# Autodesk Inventor assembly: 30-00 Injectomat suplimentar
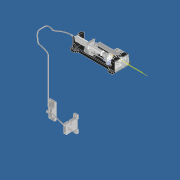
[picture p0: Inventor's stored thumbnail of the model, 180x180]
Saved by Autodesk Inventor 2020 (Build 240168000, 168)
## iProperties
Created: 2021-05-20
Part Number: 30-00 Injectomat suplimentar
Document SubType Name: Assembly
Designer: Iulian Bors
Author: Iulian Bors
## Documents named in this file (45)
- Z:\I.A.B\Proiecte\0008 I.A.B 3D 2.1 Imprimanta aracet Metal\30 Injectomat\30-00 Injectomat suplimentar.iam
- Z:\I.A.B\Proiecte\0008 I.A.B 3D 2.1 Imprimanta aracet Metal\30 Injectomat\syringe-100ml-1.snapshot.1\Corp.ipt
- Z:\I.A.B\Proiecte\0008 I.A.B 3D 2.1 Imprimanta aracet Metal\30 Injectomat\syringe-100ml-1.snapshot.1\Cauciuc.ipt
- Z:\I.A.B\Proiecte\0008 I.A.B 3D 2.1 Imprimanta aracet Metal\30 Injectomat\syringe-100ml-1.snapshot.1\Syringe_100ml.ipt
- Z:\I.A.B\Proiecte\0008 I.A.B 3D 2.1 Imprimanta aracet Metal\30 Injectomat\0008-30-002 Corp_Injectomat1.ipt
- Z:\I.A.B\Proiecte\0008 I.A.B 3D 2.1 Imprimanta aracet Metal\30 Injectomat\0008-30-001.ipt
- Z:\I.A.B\Proiecte\0008 I.A.B 3D 2.1 Imprimanta aracet Metal\30 Injectomat\0008-30-004.ipt
- Z:\I.A.B\Proiecte\0008 I.A.B 3D 2.1 Imprimanta aracet Metal\30 Injectomat\0008-30-1000 LMK8LUU.ipt
- Z:\I.A.B\Proiecte\0008 I.A.B 3D 2.1 Imprimanta aracet Metal\30 Injectomat\0008-30-1007 Bara 8.ipt
- Z:\I.A.B\Proiecte\0008 I.A.B 3D 2.1 Imprimanta aracet Metal\30 Injectomat\0008-30-1006 SHF8.ipt
- Z:\I.A.B\Proiecte\0008 I.A.B 3D 2.1 Imprimanta aracet Metal\30 Injectomat\0008-30-005.ipt
- Z:\I.A.B\Proiecte\0008 I.A.B 3D 2.1 Imprimanta aracet Metal\30 Injectomat\0008-30-1001 NEMA17 - Motor de passo.ipt
- Z:\I.A.B\Proiecte\0008 I.A.B 3D 2.1 Imprimanta aracet Metal\30 Injectomat\0008-30-1004 Piulita.ipt
- Z:\I.A.B\Proiecte\0008 I.A.B 3D 2.1 Imprimanta aracet Metal\30 Injectomat\0008-30-1003 T8 screw.ipt
- Z:\I.A.B\Proiecte\0008 I.A.B 3D 2.1 Imprimanta aracet Metal\30 Injectomat\0008-30-015 roata condusa GT2.ipt
- Z:\I.A.B\Proiecte\0008 I.A.B 3D 2.1 Imprimanta aracet Metal\30 Injectomat\0008-30-1011 GT2 Timing Pulley 20 Tooth.ipt
- Z:\I.A.B\Proiecte\0008 I.A.B 3D 2.1 Imprimanta aracet Metal\30 Injectomat\0008-30-1012 16T W6 B3 Without T_Shrinkwrap_1.ipt
- Z:\I.A.B\Proiecte\0008 I.A.B 3D 2.1 Imprimanta aracet Metal\30 Injectomat\0008-30-006.ipt
- Z:\I.A.B\Proiecte\0008 I.A.B 3D 2.1 Imprimanta aracet Metal\30 Injectomat\0008-30-1005 ISO 1224-1 - 10 - 8 x 22 x 7.ipt
- Z:\I.A.B\Proiecte\0008 I.A.B 3D 2.1 Imprimanta aracet Metal\30 Injectomat\I.A.B 2.1 Aracet_Subansamble_Shrinkwrap_2.ipt
- Z:\I.A.B\Proiecte\0008 I.A.B 3D 2.1 Imprimanta aracet Metal\30 Injectomat\0008-30-007.ipt
- Z:\I.A.B\Proiecte\0008 I.A.B 3D 2.1 Imprimanta aracet Metal\30 Injectomat\0008-30-008.ipt
- Z:\I.A.B\Proiecte\0008 I.A.B 3D 2.1 Imprimanta aracet Metal\30 Injectomat\0008-30-2002 DIN 125 - A 4.3.ipt
- Z:\I.A.B\Proiecte\0008 I.A.B 3D 2.1 Imprimanta aracet Metal\30 Injectomat\0008-30-2019 DIN 6912 - M4 x 50.ipt
- Z:\I.A.B\Proiecte\0008 I.A.B 3D 2.1 Imprimanta aracet Metal\30 Injectomat\0008-30-009.ipt
- Z:\I.A.B\Proiecte\0008 I.A.B 3D 2.1 Imprimanta aracet Metal\30 Injectomat\0008-30-2016 DIN 315 - M4.ipt
- Z:\I.A.B\Proiecte\0008 I.A.B 3D 2.1 Imprimanta aracet Metal\30 Injectomat\0008-30-010.ipt
- Z:\I.A.B\Proiecte\0008 I.A.B 3D 2.1 Imprimanta aracet Metal\30 Injectomat\0008-30-011.ipt
- Z:\I.A.B\Proiecte\0008 I.A.B 3D 2.1 Imprimanta aracet Metal\30 Injectomat\0008-30-1008 Adaptor furtun.ipt
- Z:\I.A.B\Proiecte\0008 I.A.B 3D 2.1 Imprimanta aracet Metal\30 Injectomat\0008-30-012.ipt
- Z:\I.A.B\Proiecte\0008 I.A.B 3D 2.1 Imprimanta aracet Metal\30 Injectomat\0008-30-1009 Adaptor Ac.ipt
- Z:\I.A.B\Proiecte\0008 I.A.B 3D 2.1 Imprimanta aracet Metal\30 Injectomat\0008-30-013.ipt
- Z:\I.A.B\Proiecte\0008 I.A.B 3D 2.1 Imprimanta aracet Metal\30 Injectomat\0008-30-014.ipt
- Z:\I.A.B\Proiecte\0008 I.A.B 3D 2.1 Imprimanta aracet Metal\10 Mecanic\Seringa\syringe-57.snapshot.2\SYRINGE (INVENTOR)\Needle.ipt
- Z:\I.A.B\Proiecte\0008 I.A.B 3D 2.1 Imprimanta aracet Metal\30 Injectomat\0008-30-2001 DIN 934 - M4 x 0.7.ipt
- Z:\I.A.B\Proiecte\0008 I.A.B 3D 2.1 Imprimanta aracet Metal\30 Injectomat\0008-30-203 DIN 7991 - M4x20.ipt
- Z:\I.A.B\Proiecte\0008 I.A.B 3D 2.1 Imprimanta aracet Metal\10 Mecanic\m3X16.iam
- Z:\I.A.B\Proiecte\0008 I.A.B 3D 2.1 Imprimanta aracet Metal\10 Mecanic\0008-10-2008 DIN 912 - M3 x 0.5 x 25 x 18.ipt
- Z:\I.A.B\Proiecte\0008 I.A.B 3D 2.1 Imprimanta aracet Metal\10 Mecanic\0008-10-2005 DIN 125 - A 3.2.ipt
- Z:\I.A.B\Proiecte\0008 I.A.B 3D 2.1 Imprimanta aracet Metal\10 Mecanic\0008-10-2009 DIN 555-5 - M3.ipt
- Z:\I.A.B\Proiecte\0008 I.A.B 3D 2.1 Imprimanta aracet Metal\10 Mecanic\0008-10-2004 DIN 7984 - M3 x 20.ipt
- Z:\I.A.B\Proiecte\0008 I.A.B 3D 2.1 Imprimanta aracet Metal\10 Mecanic\0008-10-2006 DIN 7984 - M3 x 16.ipt
- Z:\I.A.B\Proiecte\0008 I.A.B 3D 2.1 Imprimanta aracet Metal\30 Injectomat\30-00 Injectomat suplimentar\Design Accelerator\Synchronous Belts Transmission2.iam
- Z:\I.A.B\Proiecte\0008 I.A.B 3D 2.1 Imprimanta aracet Metal\10 Mecanic\SurubM4x25.iam
- Z:\I.A.B\Proiecte\0008 I.A.B 3D 2.1 Imprimanta aracet Metal\30 Injectomat\0008-30-2030 DIN EN ISO 4029 - M4  x  5.ipt
## Components (148 placed, 44 different names)
1. Corp.ipt:1 — Mate:1, Flush:3, Mate:18, Tangent:1, Insert:15
2. Cauciuc.ipt:2 — Insert:1, Mate:1, Mate:17
3. Syringe_100ml.ipt:3 — Insert:1, Angle:1, Mate:4, Mate:5
4. 0008-30-002 Corp_Injectomat1.ipt:4 — Angle:2, Angle:3, Angle:4, Angle:6, Mate:10, Mate:12, Mate:18, Mate:27, Tangent:1, Mate:34, Flush:8, Mate:38, Insert:6, Mate:44, Mate:45, Mate:46, Mate:47, Mate:48, Flush:10, Flush:18, Insert:27, Insert:38, Insert:39, Insert:40, Insert:41, Insert:42, Tangent:2, Insert:99, Insert:100, Insert:103, Insert:104
5. 0008-30-001.ipt:5 — Angle:3, Angle:4, Insert:3, Mate:20, Flush:6, Flush:7, Mate:21, Mate:23, Mate:24, Mate:25, Insert:64, Insert:74, Insert:75, Insert:76
6. 0008-30-004.ipt:6 — Insert:3, Mate:4, Mate:5
7. 0008-30-1000 LMK8LUU.ipt:7 — Mate:8, Mate:19, Flush:5, Flush:6, Flush:7, Mate:25, Insert:116, Insert:117, Insert:118, Insert:119
8. 0008-30-1000 LMK8LUU.ipt:8 — Mate:9, Mate:19, Mate:20, Flush:5, Insert:120, Insert:121, Insert:122, Insert:124
9. 0008-30-1007 Bara 8.ipt:9 — Mate:8, Flush:2, Mate:39, Mate:41
10. 0008-30-1007 Bara 8.ipt:10 — Mate:9, Flush:1, Mate:33, Mate:42
11. 0008-30-1006 SHF8.ipt:11 — Angle:6, Flush:2, Mate:38, Mate:39, Insert:60, Insert:93, Insert:94
12. 0008-30-1006 SHF8.ipt:12 — Flush:1, Mate:33, Mate:34, Insert:56, Insert:95, Insert:96
13. 0008-30-005.ipt:13 — Mate:10, Flush:3, Mate:17, Mate:43, Insert:10, Insert:13
14. I.A.B 2.1 Aracet_Subansamble_Shrinkwrap_2.ipt:14 — Mate:49, Flush:11, Mate:50, Flush:16, Flush:17, Flush:18, Mate:52
15. 0008-30-1001 NEMA17 - Motor de passo.ipt:15 — Mate:12, Insert:4, Flush:8, Tangent:2, Insert:86, Insert:90, Insert:91, Insert:92
16. 0008-30-1004 Piulita.ipt:16 — Mate:21, Mate:22, Mate:23, Mate:24, Insert:78, Insert:82, Insert:83, Insert:84
17. 0008-30-1003 T8 screw.ipt:17 — Mate:22, Mate:26, Flush:9, Insert:5, Mate:59
18. 0008-30-015 roata condusa GT2.ipt:18 — Mate:26, Mate:27, Flush:9, Mate:56
19. 0008-30-1011 GT2 Timing Pulley 20 Tooth.ipt:19 — Insert:4, Mate:55, Mate:57
20. 0008-30-1012 16T W6 B3 Without T_Shrinkwrap_1.ipt:20 — Mate:53, Mate:54
21. 0008-30-006.ipt:21 — Mate:41, Mate:42, Mate:43, Insert:49, Insert:50, Insert:51, Insert:52
22. 0008-30-1005 ISO 1224-1 - 10 - 8 x 22 x 7.ipt:22 — Insert:5, Insert:14
23. 0008-30-1005 ISO 1224-1 - 10 - 8 x 22 x 7.ipt:23 — Insert:6, Insert:8
24. 0008-30-007.ipt:24 — Mate:53, Mate:54
25. 0008-30-008.ipt:25 — Insert:8, Mate:58
26. 0008-30-2002 DIN 125 - A 4.3.ipt:26 — Insert:9, Insert:10
27. 0008-30-2019 DIN 6912 - M4 x 50.ipt:27 — Insert:9, Insert:12
28. 0008-30-009.ipt:28 — Insert:13
29. 0008-30-2016 DIN 315 - M4.ipt:29 — Insert:12
30. 0008-30-008.ipt:30 — Insert:14
31. 0008-30-010.ipt:31 — Mate:44, Mate:45, Mate:46
32. 0008-30-011.ipt:32 — Mate:47, Mate:48, Flush:10
33. 0008-30-2002 DIN 125 - A 4.3.ipt:33 — Insert:17, Insert:20
34. 0008-30-1008 Adaptor furtun.ipt:34 — Insert:15
35. 0008-30-012.ipt:35 — Mate:49, Flush:11, Flush:12, Flush:13, Mate:51, Flush:14, Flush:15
36. 0008-30-1009 Adaptor Ac.ipt:36 — Flush:12, Mate:50, Flush:13, Insert:16
37. 0008-30-013.ipt:37 — Mate:51, Flush:14, Flush:15, Insert:20, Insert:24
38. 0008-30-014.ipt:38 — Flush:16, Flush:17, Mate:52
39. Needle.ipt:39 — Insert:16
40. 0008-30-2001 DIN 934 - M4 x 0.7.ipt:40 — Insert:18, Insert:19
41. 0008-30-2019 DIN 6912 - M4 x 50.ipt:41 — Insert:17, Insert:19
42. 0008-30-2002 DIN 125 - A 4.3.ipt:42 — Insert:18
43. 0008-30-2001 DIN 934 - M4 x 0.7.ipt:43
44. 0008-30-2002 DIN 125 - A 4.3.ipt:44 — Insert:24
45. 0008-30-2019 DIN 6912 - M4 x 50.ipt:45
46. 0008-30-2002 DIN 125 - A 4.3.ipt:46
47. 0008-30-203 DIN 7991 - M4x20.ipt:47 — Insert:26, Insert:27
48. 0008-30-2001 DIN 934 - M4 x 0.7.ipt:48 — Insert:26
49. 0008-30-2002 DIN 125 - A 4.3.ipt:49
50. 0008-30-203 DIN 7991 - M4x20.ipt:50 — Insert:42
51. 0008-30-2001 DIN 934 - M4 x 0.7.ipt:51
52. 0008-30-2002 DIN 125 - A 4.3.ipt:52
53. 0008-30-203 DIN 7991 - M4x20.ipt:53 — Insert:41
54. 0008-30-2001 DIN 934 - M4 x 0.7.ipt:54
55. 0008-30-2002 DIN 125 - A 4.3.ipt:55
56. 0008-30-203 DIN 7991 - M4x20.ipt:56 — Insert:40
57. 0008-30-2001 DIN 934 - M4 x 0.7.ipt:57
58. 0008-30-2002 DIN 125 - A 4.3.ipt:58
59. 0008-30-203 DIN 7991 - M4x20.ipt:59 — Insert:38
60. 0008-30-2001 DIN 934 - M4 x 0.7.ipt:60
61. 0008-30-2002 DIN 125 - A 4.3.ipt:61
62. 0008-30-203 DIN 7991 - M4x20.ipt:62 — Insert:39
63. 0008-30-2001 DIN 934 - M4 x 0.7.ipt:63
64. 0008-30-2002 DIN 125 - A 4.3.ipt:64
65. 0008-30-2001 DIN 934 - M4 x 0.7.ipt:65
66. 0008-30-2002 DIN 125 - A 4.3.ipt:66 — Insert:50
67. 0008-30-2019 DIN 6912 - M4 x 50.ipt:67
68. 0008-30-2002 DIN 125 - A 4.3.ipt:68
69. 0008-30-2001 DIN 934 - M4 x 0.7.ipt:69
70. 0008-30-2002 DIN 125 - A 4.3.ipt:70 — Insert:49
71. 0008-30-2019 DIN 6912 - M4 x 50.ipt:71
72. 0008-30-2002 DIN 125 - A 4.3.ipt:72
73. m3X16.iam:73 [sub-assembly] — Insert:51
74. m3X16.iam:74 [sub-assembly] — Insert:52
75. 0008-10-2008 DIN 912 - M3 x 0.5 x 25 x 18.ipt:75 — Insert:53, Insert:55
76. 0008-10-2005 DIN 125 - A 3.2.ipt:76 — Insert:54
77. 0008-10-2009 DIN 555-5 - M3.ipt:77 — Insert:54, Insert:55
78. 0008-10-2005 DIN 125 - A 3.2.ipt:78 — Insert:53, Insert:56
79. 0008-10-2008 DIN 912 - M3 x 0.5 x 25 x 18.ipt:79
80. 0008-10-2005 DIN 125 - A 3.2.ipt:80
81. 0008-10-2009 DIN 555-5 - M3.ipt:81
82. 0008-10-2005 DIN 125 - A 3.2.ipt:82 — Insert:60
83. 0008-10-2009 DIN 555-5 - M3.ipt:83 — Insert:63
84. 0008-10-2005 DIN 125 - A 3.2.ipt:84
85. 0008-10-2005 DIN 125 - A 3.2.ipt:85 — Insert:62, Insert:64
86. 0008-10-2004 DIN 7984 - M3 x 20.ipt:86 — Insert:62, Insert:63
87. 0008-10-2009 DIN 555-5 - M3.ipt:87
88. 0008-10-2005 DIN 125 - A 3.2.ipt:88
89. 0008-10-2005 DIN 125 - A 3.2.ipt:89 — Insert:76
90. 0008-10-2004 DIN 7984 - M3 x 20.ipt:90
91. 0008-10-2009 DIN 555-5 - M3.ipt:91
92. 0008-10-2005 DIN 125 - A 3.2.ipt:92
93. 0008-10-2005 DIN 125 - A 3.2.ipt:93 — Insert:75
94. 0008-10-2004 DIN 7984 - M3 x 20.ipt:94
95. 0008-10-2009 DIN 555-5 - M3.ipt:95
96. 0008-10-2005 DIN 125 - A 3.2.ipt:96
97. 0008-10-2005 DIN 125 - A 3.2.ipt:97 — Insert:74
98. 0008-10-2004 DIN 7984 - M3 x 20.ipt:98
99. 0008-10-2006 DIN 7984 - M3 x 16.ipt:99 — Insert:78
100. 0008-10-2009 DIN 555-5 - M3.ipt:100
101. 0008-10-2006 DIN 7984 - M3 x 16.ipt:101 — Insert:82
102. 0008-10-2009 DIN 555-5 - M3.ipt:102
103. 0008-10-2006 DIN 7984 - M3 x 16.ipt:103 — Insert:83
104. 0008-10-2009 DIN 555-5 - M3.ipt:104
105. 0008-10-2006 DIN 7984 - M3 x 16.ipt:105 — Insert:84
106. 0008-10-2009 DIN 555-5 - M3.ipt:106
107. Synchronous Belts Transmission2.iam:107 [sub-assembly] — Mate:55, Mate:56, Mate:57
108. 0008-10-2006 DIN 7984 - M3 x 16.ipt:108
109. 0008-10-2005 DIN 125 - A 3.2.ipt:109 — Insert:86
110. 0008-10-2006 DIN 7984 - M3 x 16.ipt:110
111. 0008-10-2005 DIN 125 - A 3.2.ipt:111 — Insert:90
112. 0008-10-2006 DIN 7984 - M3 x 16.ipt:112
113. 0008-10-2005 DIN 125 - A 3.2.ipt:113 — Insert:92
114. 0008-10-2006 DIN 7984 - M3 x 16.ipt:114
115. 0008-10-2005 DIN 125 - A 3.2.ipt:115 — Insert:91
116. SurubM4x25.iam:116 [sub-assembly] — Insert:93
117. SurubM4x25.iam:117 [sub-assembly] — Insert:95
118. SurubM4x25.iam:118 [sub-assembly] — Insert:94
119. SurubM4x25.iam:119 [sub-assembly] — Insert:96
120. 0008-10-2005 DIN 125 - A 3.2.ipt:120 — Insert:99
121. 0008-10-2004 DIN 7984 - M3 x 20.ipt:121 — Insert:107
122. 0008-10-2005 DIN 125 - A 3.2.ipt:122 — Insert:100
123. 0008-10-2004 DIN 7984 - M3 x 20.ipt:123 — Insert:108
124. 0008-10-2009 DIN 555-5 - M3.ipt:124
125. 0008-10-2005 DIN 125 - A 3.2.ipt:125 — Insert:103
126. 0008-10-2009 DIN 555-5 - M3.ipt:126
127. 0008-10-2005 DIN 125 - A 3.2.ipt:127 — Insert:104
128. 0008-10-2009 DIN 555-5 - M3.ipt:128 — Insert:107
129. 0008-10-2005 DIN 125 - A 3.2.ipt:129
130. 0008-10-2009 DIN 555-5 - M3.ipt:130 — Insert:108
131. 0008-10-2005 DIN 125 - A 3.2.ipt:131
132. 0008-10-2006 DIN 7984 - M3 x 16.ipt:132 — Insert:117
133. 0008-10-2009 DIN 555-5 - M3.ipt:133
134. 0008-10-2006 DIN 7984 - M3 x 16.ipt:134 — Insert:118
135. 0008-10-2009 DIN 555-5 - M3.ipt:135
136. 0008-10-2006 DIN 7984 - M3 x 16.ipt:136 — Insert:119
137. 0008-10-2009 DIN 555-5 - M3.ipt:137
138. 0008-10-2006 DIN 7984 - M3 x 16.ipt:138 — Insert:121
139. 0008-10-2009 DIN 555-5 - M3.ipt:139
140. 0008-10-2006 DIN 7984 - M3 x 16.ipt:140 — Insert:122
141. 0008-10-2009 DIN 555-5 - M3.ipt:141
142. 0008-10-2006 DIN 7984 - M3 x 16.ipt:142 — Insert:120
143. 0008-10-2009 DIN 555-5 - M3.ipt:143
144. 0008-10-2006 DIN 7984 - M3 x 16.ipt:144 — Insert:116
145. 0008-10-2009 DIN 555-5 - M3.ipt:145
146. 0008-10-2006 DIN 7984 - M3 x 16.ipt:146 — Insert:124
147. 0008-10-2009 DIN 555-5 - M3.ipt:147
148. 0008-30-2030 DIN EN ISO 4029 - M4  x  5.ipt:148 — Mate:58, Mate:59
## Relationships (188: Insert 121, Mate 42, Flush 18, Angle 5, Tangent 2)
- Insert:1: Cauciuc.ipt:2 ↔ Syringe_100ml.ipt:3
- Mate:1: Corp.ipt:1 ↔ Cauciuc.ipt:2
- Angle:1 (0 deg): Syringe_100ml.ipt:3
- Angle:2 (180 deg): 0008-30-002 Corp_Injectomat1.ipt:4
- Angle:3 (180 deg): 0008-30-002 Corp_Injectomat1.ipt:4 ↔ 0008-30-001.ipt:5
- Angle:4 (180 deg): 0008-30-002 Corp_Injectomat1.ipt:4 ↔ 0008-30-001.ipt:5
- Insert:3: 0008-30-001.ipt:5 ↔ 0008-30-004.ipt:6
- Mate:4: Syringe_100ml.ipt:3 ↔ 0008-30-004.ipt:6
- Mate:5: Syringe_100ml.ipt:3 ↔ 0008-30-004.ipt:6
- Mate:8: 0008-30-1000 LMK8LUU.ipt:7 ↔ 0008-30-1007 Bara 8.ipt:9
- Mate:9: 0008-30-1000 LMK8LUU.ipt:8 ↔ 0008-30-1007 Bara 8.ipt:10
- Angle:6 (0 deg): 0008-30-002 Corp_Injectomat1.ipt:4 ↔ 0008-30-1006 SHF8.ipt:11
- Flush:1: 0008-30-1007 Bara 8.ipt:10 ↔ 0008-30-1006 SHF8.ipt:12
- Flush:2: 0008-30-1007 Bara 8.ipt:9 ↔ 0008-30-1006 SHF8.ipt:11
- [Flush] (30 mm): 0008-30-002 Corp_Injectomat1.ipt:4 ↔ I.A.B 2.1 Aracet_Subansamble_Shrinkwrap_2.ipt:14
- Mate:10: 0008-30-002 Corp_Injectomat1.ipt:4 ↔ 0008-30-005.ipt:13
- Flush:3 (-5 mm): Corp.ipt:1 ↔ 0008-30-005.ipt:13
- [Mate]: 0008-30-002 Corp_Injectomat1.ipt:4 ↔ I.A.B 2.1 Aracet_Subansamble_Shrinkwrap_2.ipt:14
- Mate:12: 0008-30-002 Corp_Injectomat1.ipt:4 ↔ 0008-30-1001 NEMA17 - Motor de passo.ipt:15
- Mate:17: Cauciuc.ipt:2 ↔ 0008-30-005.ipt:13
- Mate:18: Corp.ipt:1 ↔ 0008-30-002 Corp_Injectomat1.ipt:4
- Mate:19 (3 mm): 0008-30-1000 LMK8LUU.ipt:7 ↔ 0008-30-1000 LMK8LUU.ipt:8
- Mate:20: 0008-30-001.ipt:5 ↔ 0008-30-1000 LMK8LUU.ipt:8
- Flush:5: 0008-30-1000 LMK8LUU.ipt:7 ↔ 0008-30-1000 LMK8LUU.ipt:8
- Flush:6 (5 mm): 0008-30-001.ipt:5 ↔ 0008-30-1000 LMK8LUU.ipt:7
- Flush:7 (40 mm): 0008-30-001.ipt:5 ↔ 0008-30-1000 LMK8LUU.ipt:7
- Mate:21: 0008-30-001.ipt:5 ↔ 0008-30-1004 Piulita.ipt:16
- Mate:22: 0008-30-1004 Piulita.ipt:16 ↔ 0008-30-1003 T8 screw.ipt:17
- Mate:23: 0008-30-001.ipt:5 ↔ 0008-30-1004 Piulita.ipt:16
- Mate:24: 0008-30-001.ipt:5 ↔ 0008-30-1004 Piulita.ipt:16
- Mate:25: 0008-30-001.ipt:5 ↔ 0008-30-1000 LMK8LUU.ipt:7
- Mate:26: 0008-30-1003 T8 screw.ipt:17 ↔ 0008-30-015 roata condusa GT2.ipt:18
- Mate:27 (1 mm): 0008-30-002 Corp_Injectomat1.ipt:4 ↔ 0008-30-015 roata condusa GT2.ipt:18
- Tangent:1 (-0.5 mm): Corp.ipt:1 ↔ 0008-30-002 Corp_Injectomat1.ipt:4
- Insert:4 (2 mm): 0008-30-1001 NEMA17 - Motor de passo.ipt:15 ↔ 0008-30-1011 GT2 Timing Pulley 20 Tooth.ipt:19
- Mate:33: 0008-30-1007 Bara 8.ipt:10 ↔ 0008-30-1006 SHF8.ipt:12
- Mate:34: 0008-30-002 Corp_Injectomat1.ipt:4 ↔ 0008-30-1006 SHF8.ipt:12
- Flush:8 (1 mm): 0008-30-002 Corp_Injectomat1.ipt:4 ↔ 0008-30-1001 NEMA17 - Motor de passo.ipt:15
- Mate:38: 0008-30-002 Corp_Injectomat1.ipt:4 ↔ 0008-30-1006 SHF8.ipt:11
- Mate:39: 0008-30-1007 Bara 8.ipt:9 ↔ 0008-30-1006 SHF8.ipt:11
- Flush:9: 0008-30-1003 T8 screw.ipt:17 ↔ 0008-30-015 roata condusa GT2.ipt:18
- Mate:41: 0008-30-1007 Bara 8.ipt:9 ↔ 0008-30-006.ipt:21
- Mate:42: 0008-30-1007 Bara 8.ipt:10 ↔ 0008-30-006.ipt:21
- Mate:43: 0008-30-005.ipt:13 ↔ 0008-30-006.ipt:21
- Insert:5: 0008-30-1003 T8 screw.ipt:17 ↔ 0008-30-1005 ISO 1224-1 - 10 - 8 x 22 x 7.ipt:22
- Insert:6: 0008-30-002 Corp_Injectomat1.ipt:4 ↔ 0008-30-1005 ISO 1224-1 - 10 - 8 x 22 x 7.ipt:23
- Insert:8: 0008-30-1005 ISO 1224-1 - 10 - 8 x 22 x 7.ipt:23 ↔ 0008-30-008.ipt:25
- Insert:9: 0008-30-2002 DIN 125 - A 4.3.ipt:26 ↔ 0008-30-2019 DIN 6912 - M4 x 50.ipt:27
- Insert:10: 0008-30-005.ipt:13 ↔ 0008-30-2002 DIN 125 - A 4.3.ipt:26
- Insert:12: 0008-30-2019 DIN 6912 - M4 x 50.ipt:27 ↔ 0008-30-2016 DIN 315 - M4.ipt:29
- Insert:13: 0008-30-005.ipt:13 ↔ 0008-30-009.ipt:28
- Insert:14: 0008-30-1005 ISO 1224-1 - 10 - 8 x 22 x 7.ipt:22 ↔ 0008-30-008.ipt:30
- Mate:44: 0008-30-002 Corp_Injectomat1.ipt:4 ↔ 0008-30-010.ipt:31
- Mate:45 (1 mm): 0008-30-002 Corp_Injectomat1.ipt:4 ↔ 0008-30-010.ipt:31
- Mate:46 (1 mm): 0008-30-002 Corp_Injectomat1.ipt:4 ↔ 0008-30-010.ipt:31
- Mate:47: 0008-30-002 Corp_Injectomat1.ipt:4 ↔ 0008-30-011.ipt:32
- Mate:48: 0008-30-002 Corp_Injectomat1.ipt:4 ↔ 0008-30-011.ipt:32
- Flush:10: 0008-30-002 Corp_Injectomat1.ipt:4 ↔ 0008-30-011.ipt:32
- Insert:15: Corp.ipt:1 ↔ 0008-30-1008 Adaptor furtun.ipt:34
- Mate:49: I.A.B 2.1 Aracet_Subansamble_Shrinkwrap_2.ipt:14 ↔ 0008-30-012.ipt:35
- Flush:11: I.A.B 2.1 Aracet_Subansamble_Shrinkwrap_2.ipt:14 ↔ 0008-30-012.ipt:35
- Flush:12 (-2 mm): 0008-30-012.ipt:35 ↔ 0008-30-1009 Adaptor Ac.ipt:36
- Mate:50 (77 mm): I.A.B 2.1 Aracet_Subansamble_Shrinkwrap_2.ipt:14 ↔ 0008-30-1009 Adaptor Ac.ipt:36
- Flush:13: 0008-30-012.ipt:35 ↔ 0008-30-1009 Adaptor Ac.ipt:36
- Mate:51 (2 mm): 0008-30-012.ipt:35 ↔ 0008-30-013.ipt:37
- Flush:14: 0008-30-012.ipt:35 ↔ 0008-30-013.ipt:37
- Flush:15: 0008-30-012.ipt:35 ↔ 0008-30-013.ipt:37
- Flush:16: I.A.B 2.1 Aracet_Subansamble_Shrinkwrap_2.ipt:14 ↔ 0008-30-014.ipt:38
- Flush:17: I.A.B 2.1 Aracet_Subansamble_Shrinkwrap_2.ipt:14 ↔ 0008-30-014.ipt:38
- Flush:18 (-2 mm): 0008-30-002 Corp_Injectomat1.ipt:4 ↔ I.A.B 2.1 Aracet_Subansamble_Shrinkwrap_2.ipt:14
- Mate:52: I.A.B 2.1 Aracet_Subansamble_Shrinkwrap_2.ipt:14 ↔ 0008-30-014.ipt:38
- Insert:16 (-5 mm): 0008-30-1009 Adaptor Ac.ipt:36 ↔ Needle.ipt:39
- Mate:53: 0008-30-1012 16T W6 B3 Without T_Shrinkwrap_1.ipt:20 ↔ 0008-30-007.ipt:24
- Mate:54: 0008-30-1012 16T W6 B3 Without T_Shrinkwrap_1.ipt:20 ↔ 0008-30-007.ipt:24
- Insert:17: 0008-30-2002 DIN 125 - A 4.3.ipt:33 ↔ 0008-30-2019 DIN 6912 - M4 x 50.ipt:41
- Insert:18: 0008-30-2001 DIN 934 - M4 x 0.7.ipt:40 ↔ 0008-30-2002 DIN 125 - A 4.3.ipt:42
- Insert:19: 0008-30-2001 DIN 934 - M4 x 0.7.ipt:40 ↔ 0008-30-2019 DIN 6912 - M4 x 50.ipt:41
- Insert:20: 0008-30-2002 DIN 125 - A 4.3.ipt:33 ↔ 0008-30-013.ipt:37
- [Insert]: 0008-30-2002 DIN 125 - A 4.3.ipt:44 ↔ 0008-30-2019 DIN 6912 - M4 x 50.ipt:45
- [Insert]: 0008-30-2001 DIN 934 - M4 x 0.7.ipt:43 ↔ 0008-30-2002 DIN 125 - A 4.3.ipt:46
- [Insert]: 0008-30-2001 DIN 934 - M4 x 0.7.ipt:43 ↔ 0008-30-2019 DIN 6912 - M4 x 50.ipt:45
- Insert:24: 0008-30-013.ipt:37 ↔ 0008-30-2002 DIN 125 - A 4.3.ipt:44
- [Insert]: 0008-30-2001 DIN 934 - M4 x 0.7.ipt:48 ↔ 0008-30-2002 DIN 125 - A 4.3.ipt:49
- Insert:26: 0008-30-203 DIN 7991 - M4x20.ipt:47 ↔ 0008-30-2001 DIN 934 - M4 x 0.7.ipt:48
- Insert:27: 0008-30-002 Corp_Injectomat1.ipt:4 ↔ 0008-30-203 DIN 7991 - M4x20.ipt:47
- [Insert]: 0008-30-2001 DIN 934 - M4 x 0.7.ipt:51 ↔ 0008-30-2002 DIN 125 - A 4.3.ipt:52
- [Insert]: 0008-30-203 DIN 7991 - M4x20.ipt:50 ↔ 0008-30-2001 DIN 934 - M4 x 0.7.ipt:51
- [Insert]: 0008-30-2001 DIN 934 - M4 x 0.7.ipt:54 ↔ 0008-30-2002 DIN 125 - A 4.3.ipt:55
- [Insert]: 0008-30-203 DIN 7991 - M4x20.ipt:53 ↔ 0008-30-2001 DIN 934 - M4 x 0.7.ipt:54
- [Insert]: 0008-30-2001 DIN 934 - M4 x 0.7.ipt:57 ↔ 0008-30-2002 DIN 125 - A 4.3.ipt:58
- [Insert]: 0008-30-203 DIN 7991 - M4x20.ipt:56 ↔ 0008-30-2001 DIN 934 - M4 x 0.7.ipt:57
- [Insert]: 0008-30-2001 DIN 934 - M4 x 0.7.ipt:60 ↔ 0008-30-2002 DIN 125 - A 4.3.ipt:61
- [Insert]: 0008-30-203 DIN 7991 - M4x20.ipt:59 ↔ 0008-30-2001 DIN 934 - M4 x 0.7.ipt:60
- [Insert]: 0008-30-2001 DIN 934 - M4 x 0.7.ipt:63 ↔ 0008-30-2002 DIN 125 - A 4.3.ipt:64
- [Insert]: 0008-30-203 DIN 7991 - M4x20.ipt:62 ↔ 0008-30-2001 DIN 934 - M4 x 0.7.ipt:63
- Insert:38: 0008-30-002 Corp_Injectomat1.ipt:4 ↔ 0008-30-203 DIN 7991 - M4x20.ipt:59
- Insert:39: 0008-30-002 Corp_Injectomat1.ipt:4 ↔ 0008-30-203 DIN 7991 - M4x20.ipt:62
- Insert:40: 0008-30-002 Corp_Injectomat1.ipt:4 ↔ 0008-30-203 DIN 7991 - M4x20.ipt:56
- Insert:41: 0008-30-002 Corp_Injectomat1.ipt:4 ↔ 0008-30-203 DIN 7991 - M4x20.ipt:53
- Insert:42: 0008-30-002 Corp_Injectomat1.ipt:4 ↔ 0008-30-203 DIN 7991 - M4x20.ipt:50
- [Insert]: 0008-30-2002 DIN 125 - A 4.3.ipt:66 ↔ 0008-30-2019 DIN 6912 - M4 x 50.ipt:67
- [Insert]: 0008-30-2001 DIN 934 - M4 x 0.7.ipt:65 ↔ 0008-30-2002 DIN 125 - A 4.3.ipt:68
- [Insert]: 0008-30-2001 DIN 934 - M4 x 0.7.ipt:65 ↔ 0008-30-2019 DIN 6912 - M4 x 50.ipt:67
- [Insert]: 0008-30-2002 DIN 125 - A 4.3.ipt:70 ↔ 0008-30-2019 DIN 6912 - M4 x 50.ipt:71
- [Insert]: 0008-30-2001 DIN 934 - M4 x 0.7.ipt:69 ↔ 0008-30-2002 DIN 125 - A 4.3.ipt:72
- [Insert]: 0008-30-2001 DIN 934 - M4 x 0.7.ipt:69 ↔ 0008-30-2019 DIN 6912 - M4 x 50.ipt:71
- Insert:49: 0008-30-006.ipt:21 ↔ 0008-30-2002 DIN 125 - A 4.3.ipt:70
- Insert:50: 0008-30-006.ipt:21 ↔ 0008-30-2002 DIN 125 - A 4.3.ipt:66
- Insert:51: 0008-30-006.ipt:21 ↔ m3X16.iam:73
- Insert:52: 0008-30-006.ipt:21 ↔ m3X16.iam:74
- Insert:53: 0008-10-2008 DIN 912 - M3 x 0.5 x 25 x 18.ipt:75 ↔ 0008-10-2005 DIN 125 - A 3.2.ipt:78
- Insert:54: 0008-10-2005 DIN 125 - A 3.2.ipt:76 ↔ 0008-10-2009 DIN 555-5 - M3.ipt:77
- Insert:55: 0008-10-2008 DIN 912 - M3 x 0.5 x 25 x 18.ipt:75 ↔ 0008-10-2009 DIN 555-5 - M3.ipt:77
- Insert:56: 0008-30-1006 SHF8.ipt:12 ↔ 0008-10-2005 DIN 125 - A 3.2.ipt:78
- [Insert]: 0008-10-2008 DIN 912 - M3 x 0.5 x 25 x 18.ipt:79 ↔ 0008-10-2005 DIN 125 - A 3.2.ipt:82
- [Insert]: 0008-10-2005 DIN 125 - A 3.2.ipt:80 ↔ 0008-10-2009 DIN 555-5 - M3.ipt:81
- [Insert]: 0008-10-2008 DIN 912 - M3 x 0.5 x 25 x 18.ipt:79 ↔ 0008-10-2009 DIN 555-5 - M3.ipt:81
- Insert:60: 0008-30-1006 SHF8.ipt:11 ↔ 0008-10-2005 DIN 125 - A 3.2.ipt:82
- [Insert]: 0008-10-2009 DIN 555-5 - M3.ipt:83 ↔ 0008-10-2005 DIN 125 - A 3.2.ipt:84
- Insert:62: 0008-10-2005 DIN 125 - A 3.2.ipt:85 ↔ 0008-10-2004 DIN 7984 - M3 x 20.ipt:86
- Insert:63 (-0.5 mm): 0008-10-2009 DIN 555-5 - M3.ipt:83 ↔ 0008-10-2004 DIN 7984 - M3 x 20.ipt:86
- Insert:64: 0008-30-001.ipt:5 ↔ 0008-10-2005 DIN 125 - A 3.2.ipt:85
- [Insert]: 0008-10-2009 DIN 555-5 - M3.ipt:87 ↔ 0008-10-2005 DIN 125 - A 3.2.ipt:88
- [Insert]: 0008-10-2005 DIN 125 - A 3.2.ipt:89 ↔ 0008-10-2004 DIN 7984 - M3 x 20.ipt:90
- [Insert] (-0.5 mm): 0008-10-2009 DIN 555-5 - M3.ipt:87 ↔ 0008-10-2004 DIN 7984 - M3 x 20.ipt:90
- [Insert]: 0008-10-2009 DIN 555-5 - M3.ipt:91 ↔ 0008-10-2005 DIN 125 - A 3.2.ipt:92
- [Insert]: 0008-10-2005 DIN 125 - A 3.2.ipt:93 ↔ 0008-10-2004 DIN 7984 - M3 x 20.ipt:94
- [Insert] (-0.5 mm): 0008-10-2009 DIN 555-5 - M3.ipt:91 ↔ 0008-10-2004 DIN 7984 - M3 x 20.ipt:94
- [Insert]: 0008-10-2009 DIN 555-5 - M3.ipt:95 ↔ 0008-10-2005 DIN 125 - A 3.2.ipt:96
- [Insert]: 0008-10-2005 DIN 125 - A 3.2.ipt:97 ↔ 0008-10-2004 DIN 7984 - M3 x 20.ipt:98
- [Insert] (-0.5 mm): 0008-10-2009 DIN 555-5 - M3.ipt:95 ↔ 0008-10-2004 DIN 7984 - M3 x 20.ipt:98
- Insert:74: 0008-30-001.ipt:5 ↔ 0008-10-2005 DIN 125 - A 3.2.ipt:97
- Insert:75: 0008-30-001.ipt:5 ↔ 0008-10-2005 DIN 125 - A 3.2.ipt:93
- Insert:76: 0008-30-001.ipt:5 ↔ 0008-10-2005 DIN 125 - A 3.2.ipt:89
- [Insert]: 0008-10-2006 DIN 7984 - M3 x 16.ipt:99 ↔ 0008-10-2009 DIN 555-5 - M3.ipt:100
- Insert:78: 0008-30-1004 Piulita.ipt:16 ↔ 0008-10-2006 DIN 7984 - M3 x 16.ipt:99
- [Insert]: 0008-10-2006 DIN 7984 - M3 x 16.ipt:101 ↔ 0008-10-2009 DIN 555-5 - M3.ipt:102
- [Insert]: 0008-10-2006 DIN 7984 - M3 x 16.ipt:103 ↔ 0008-10-2009 DIN 555-5 - M3.ipt:104
- [Insert]: 0008-10-2006 DIN 7984 - M3 x 16.ipt:105 ↔ 0008-10-2009 DIN 555-5 - M3.ipt:106
- Insert:82: 0008-30-1004 Piulita.ipt:16 ↔ 0008-10-2006 DIN 7984 - M3 x 16.ipt:101
- Insert:83: 0008-30-1004 Piulita.ipt:16 ↔ 0008-10-2006 DIN 7984 - M3 x 16.ipt:103
- Insert:84: 0008-30-1004 Piulita.ipt:16 ↔ 0008-10-2006 DIN 7984 - M3 x 16.ipt:105
- Mate:55: 0008-30-1011 GT2 Timing Pulley 20 Tooth.ipt:19 ↔ Synchronous Belts Transmission2.iam:107
- Tangent:2 (0.5 mm): 0008-30-002 Corp_Injectomat1.ipt:4 ↔ 0008-30-1001 NEMA17 - Motor de passo.ipt:15
- Mate:56: 0008-30-015 roata condusa GT2.ipt:18 ↔ Synchronous Belts Transmission2.iam:107
- Mate:57 (2 mm): 0008-30-1011 GT2 Timing Pulley 20 Tooth.ipt:19 ↔ Synchronous Belts Transmission2.iam:107
- [Insert]: 0008-10-2006 DIN 7984 - M3 x 16.ipt:108 ↔ 0008-10-2005 DIN 125 - A 3.2.ipt:109
- Insert:86 (10 mm): 0008-30-1001 NEMA17 - Motor de passo.ipt:15 ↔ 0008-10-2005 DIN 125 - A 3.2.ipt:109
- [Insert]: 0008-10-2006 DIN 7984 - M3 x 16.ipt:110 ↔ 0008-10-2005 DIN 125 - A 3.2.ipt:111
- [Insert]: 0008-10-2006 DIN 7984 - M3 x 16.ipt:112 ↔ 0008-10-2005 DIN 125 - A 3.2.ipt:113
- [Insert]: 0008-10-2006 DIN 7984 - M3 x 16.ipt:114 ↔ 0008-10-2005 DIN 125 - A 3.2.ipt:115
- Insert:90 (10 mm): 0008-30-1001 NEMA17 - Motor de passo.ipt:15 ↔ 0008-10-2005 DIN 125 - A 3.2.ipt:111
- Insert:91 (10 mm): 0008-30-1001 NEMA17 - Motor de passo.ipt:15 ↔ 0008-10-2005 DIN 125 - A 3.2.ipt:115
- Insert:92 (10 mm): 0008-30-1001 NEMA17 - Motor de passo.ipt:15 ↔ 0008-10-2005 DIN 125 - A 3.2.ipt:113
- Insert:93: 0008-30-1006 SHF8.ipt:11 ↔ SurubM4x25.iam:116
- Insert:94: 0008-30-1006 SHF8.ipt:11 ↔ SurubM4x25.iam:118
- Insert:95: 0008-30-1006 SHF8.ipt:12 ↔ SurubM4x25.iam:117
- Insert:96: 0008-30-1006 SHF8.ipt:12 ↔ SurubM4x25.iam:119
- [Insert]: 0008-10-2005 DIN 125 - A 3.2.ipt:120 ↔ 0008-10-2004 DIN 7984 - M3 x 20.ipt:121
- [Insert]: 0008-10-2005 DIN 125 - A 3.2.ipt:122 ↔ 0008-10-2004 DIN 7984 - M3 x 20.ipt:123
- Insert:99: 0008-30-002 Corp_Injectomat1.ipt:4 ↔ 0008-10-2005 DIN 125 - A 3.2.ipt:120
- Insert:100: 0008-30-002 Corp_Injectomat1.ipt:4 ↔ 0008-10-2005 DIN 125 - A 3.2.ipt:122
- [Insert]: 0008-10-2009 DIN 555-5 - M3.ipt:124 ↔ 0008-10-2005 DIN 125 - A 3.2.ipt:125
- [Insert]: 0008-10-2009 DIN 555-5 - M3.ipt:126 ↔ 0008-10-2005 DIN 125 - A 3.2.ipt:127
- Insert:103: 0008-30-002 Corp_Injectomat1.ipt:4 ↔ 0008-10-2005 DIN 125 - A 3.2.ipt:125
- Insert:104: 0008-30-002 Corp_Injectomat1.ipt:4 ↔ 0008-10-2005 DIN 125 - A 3.2.ipt:127
- [Insert]: 0008-10-2009 DIN 555-5 - M3.ipt:128 ↔ 0008-10-2005 DIN 125 - A 3.2.ipt:129
- [Insert]: 0008-10-2009 DIN 555-5 - M3.ipt:130 ↔ 0008-10-2005 DIN 125 - A 3.2.ipt:131
- Insert:107 (1.5 mm): 0008-10-2004 DIN 7984 - M3 x 20.ipt:121 ↔ 0008-10-2009 DIN 555-5 - M3.ipt:128
- Insert:108 (1.5 mm): 0008-10-2004 DIN 7984 - M3 x 20.ipt:123 ↔ 0008-10-2009 DIN 555-5 - M3.ipt:130
- [Insert]: 0008-10-2006 DIN 7984 - M3 x 16.ipt:132 ↔ 0008-10-2009 DIN 555-5 - M3.ipt:133
- [Insert]: 0008-10-2006 DIN 7984 - M3 x 16.ipt:134 ↔ 0008-10-2009 DIN 555-5 - M3.ipt:135
- [Insert]: 0008-10-2006 DIN 7984 - M3 x 16.ipt:136 ↔ 0008-10-2009 DIN 555-5 - M3.ipt:137
- [Insert]: 0008-10-2006 DIN 7984 - M3 x 16.ipt:138 ↔ 0008-10-2009 DIN 555-5 - M3.ipt:139
- [Insert]: 0008-10-2006 DIN 7984 - M3 x 16.ipt:140 ↔ 0008-10-2009 DIN 555-5 - M3.ipt:141
- [Insert]: 0008-10-2006 DIN 7984 - M3 x 16.ipt:142 ↔ 0008-10-2009 DIN 555-5 - M3.ipt:143
- [Insert]: 0008-10-2006 DIN 7984 - M3 x 16.ipt:144 ↔ 0008-10-2009 DIN 555-5 - M3.ipt:145
- Insert:116: 0008-30-1000 LMK8LUU.ipt:7 ↔ 0008-10-2006 DIN 7984 - M3 x 16.ipt:144
- Insert:117: 0008-30-1000 LMK8LUU.ipt:7 ↔ 0008-10-2006 DIN 7984 - M3 x 16.ipt:132
- Insert:118: 0008-30-1000 LMK8LUU.ipt:7 ↔ 0008-10-2006 DIN 7984 - M3 x 16.ipt:134
- Insert:119: 0008-30-1000 LMK8LUU.ipt:7 ↔ 0008-10-2006 DIN 7984 - M3 x 16.ipt:136
- Insert:120: 0008-30-1000 LMK8LUU.ipt:8 ↔ 0008-10-2006 DIN 7984 - M3 x 16.ipt:142
- Insert:121: 0008-30-1000 LMK8LUU.ipt:8 ↔ 0008-10-2006 DIN 7984 - M3 x 16.ipt:138
- Insert:122: 0008-30-1000 LMK8LUU.ipt:8 ↔ 0008-10-2006 DIN 7984 - M3 x 16.ipt:140
- [Insert]: 0008-10-2006 DIN 7984 - M3 x 16.ipt:146 ↔ 0008-10-2009 DIN 555-5 - M3.ipt:147
- Insert:124: 0008-30-1000 LMK8LUU.ipt:8 ↔ 0008-10-2006 DIN 7984 - M3 x 16.ipt:146
- Mate:58: 0008-30-008.ipt:25 ↔ 0008-30-2030 DIN EN ISO 4029 - M4  x  5.ipt:148
- Mate:59 (5 mm): 0008-30-1003 T8 screw.ipt:17 ↔ 0008-30-2030 DIN EN ISO 4029 - M4  x  5.ipt:148
## Named parameters: d123_d119 = 0 mm, d124_d120 = 0 mm, d125_d121 = 0 mm, d127_d120 = 0 mm, d130_d127_d120 = 0 mm, d131_d128 = 0 mm, d132_d127_d120 = 0 mm, d133_d128 = 0 mm, d134_d127_d120 = 0 mm, d135_d128 = 0 mm, d136_d127_d120 = 0 mm, d137_d128 = 0 mm, d138_d127_d120 = 0 mm, d139_d128 = 0 mm, d145_d119 = 0 mm, d146_d120 = 0 mm, d147_d121 = 0 mm, d148_d119 = 0 mm, d149_d120 = 0 mm, d150_d121 = 0 mm, d159_d155 = 0 mm, d160_d156 = 0 mm, d161_d157 = 0 mm, d163_d2 = 0 mm, d169_d167 = -0.5 mm, d170_d163_d2 = 0 mm, d171_d166 = 0 mm, d172_d167 = -0.5 mm, d173_d163_d2 = 0 mm, d174_d166 = 0 mm, d175_d167 = -0.5 mm, d176_d163_d2 = 0 mm, d177_d166 = 0 mm, d181_d0 = 0 mm, d183_d0 = 0 mm, d184_d0 = 0 mm, d185_d0 = 0 mm, d193_d1 = 0 mm, d195_d193_d1 = 0 mm, d196_d193_d1 = 0 mm, d197_d193_d1 = 0 mm, d205_d166 = 0 mm, d206_d166 = 0 mm, d209_d176_d163_d2 = 0 mm, d210_d176_d163_d2 = 0 mm, d213_d176_d163_d2 = 0 mm, d214_d176_d163_d2 = 0 mm, d217_d181_d0 = 0 mm, d218_d181_d0 = 0 mm, d219_d181_d0 = 0 mm, d220_d181_d0 = 0 mm, d221_d181_d0 = 0 mm, d222_d181_d0 = 0 mm, d223_d181_d0 = 0 mm, d231_d181_d0 = 0 mm
